# Autodesk Inventor assembly: Assembly
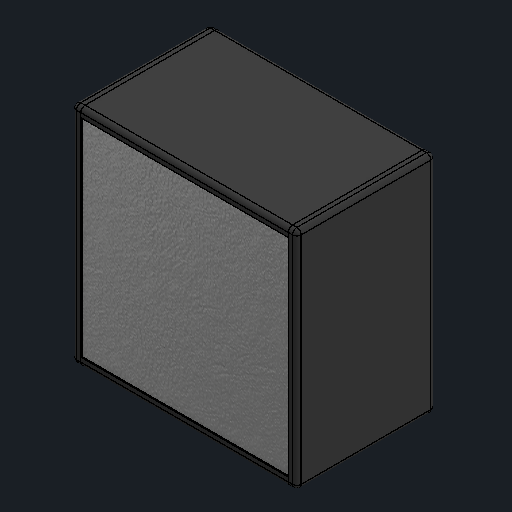
[picture p0: Inventor's stored thumbnail of the model, 512x512]
Saved by Autodesk Inventor 2026.2 (Build 302298000, 298)
## iProperties
Created: 2026-06-16
Part Number: Assembly
Document SubType Name: Assembly
Designer: JoshuaEah
Author: JoshuaEah
## Documents named in this file (18)
- C:\Users\JoshuaEah\Documents\GitHub\Designed-Trinkets\Guitar\110 Guitar Cab\Assembly.iam
- C:\Users\JoshuaEah\Documents\GitHub\Designed-Trinkets\Guitar\110 Guitar Cab\Wood Cuts\Bracing.iam
- C:\Users\JoshuaEah\Documents\GitHub\Designed-Trinkets\Guitar\110 Guitar Cab\Wood Cuts\Front Baffle.ipt
- C:\Users\JoshuaEah\Documents\GitHub\Designed-Trinkets\Guitar\110 Guitar Cab\Wood Cuts\Grille.ipt
- C:\Users\JoshuaEah\Documents\GitHub\Designed-Trinkets\Guitar\110 Guitar Cab\Sheet Metal\Jack Plate.ipt
- C:\Users\JoshuaEah\Documents\GitHub\Designed-Trinkets\Guitar\110 Guitar Cab\Hardware\Grill Cloth.ipt
- C:\Users\JoshuaEah\Documents\GitHub\Designed-Trinkets\Guitar\110 Guitar Cab\Wood Cuts\Top Panel.ipt
- C:\Users\JoshuaEah\Documents\GitHub\Designed-Trinkets\Guitar\110 Guitar Cab\Wood Cuts\Bottom Panel.ipt
- C:\Users\JoshuaEah\Documents\GitHub\Designed-Trinkets\Guitar\110 Guitar Cab\Wood Cuts\Side Panel (Right).ipt
- C:\Users\JoshuaEah\Documents\GitHub\Designed-Trinkets\Guitar\110 Guitar Cab\Wood Cuts\Side Panel (Left).ipt
- C:\Users\JoshuaEah\Documents\GitHub\Designed-Trinkets\Guitar\110 Guitar Cab\Hardware\Switchcraft C11X Jack.ipt
- C:\Users\JoshuaEah\Documents\GitHub\Designed-Trinkets\Guitar\110 Guitar Cab\Hardware\Switchcraft C11X Washer.ipt
- C:\Users\JoshuaEah\Documents\GitHub\Designed-Trinkets\Guitar\110 Guitar Cab\Hardware\Switchcraft C11X Nut.ipt
- C:\Users\JoshuaEah\Documents\GitHub\Designed-Trinkets\Guitar\110 Guitar Cab\Hardware\No. 4x1in PH1 Wood Screw.ipt
- C:\Users\JoshuaEah\Documents\GitHub\Designed-Trinkets\Guitar\110 Guitar Cab\Wood Cuts\Back Panel (Top).ipt
- C:\Users\JoshuaEah\Documents\GitHub\Designed-Trinkets\Guitar\110 Guitar Cab\Wood Cuts\Back Panel (Bottom).ipt
- C:\Users\JoshuaEah\Documents\GitHub\Designed-Trinkets\Guitar\110 Guitar Cab\Sheet Metal\Name Plate.ipt
- C:\Users\JoshuaEah\Documents\GitHub\Designed-Trinkets\Guitar\110 Guitar Cab\Hardware\No. 6-32x0.5in FHCS PH2.ipt
## Components (32 placed, 17 different names)
1. Top Panel:1 — Mate:1, Flush:1, Flush:2, Mate:2, Flush:3, Flush:4, Flush:10, Mate:16, Flush:15
2. Bottom Panel:1 — Flush:5, Flush:6, Mate:3
3. Side Panel (Right):1 — Mate:1, Flush:1, Flush:2, Flush:5, Flush:6, Mate:3, Mate:17
4. Side Panel (Left):1 — Mate:2, Flush:3, Flush:4
5. Front Baffle — Mate:20, Flush:16, Flush:17, Mate:21, Flush:18, Flush:19
6. Bracing:1 [sub-assembly] — Flush:15, Mate:20, Flush:16, Flush:17
7. Bracing:2 [sub-assembly] — Flush:10, Mate:16, Mate:17, Mate:18, Flush:11, Flush:12, Mate:19, Flush:13, Flush:14
8. Back Panel (Top):1 — Mate:18, Flush:11, Flush:12, Insert:8, Insert:12, Insert:13
9. Jack Plate:1 — Insert:3, Insert:4, Insert:14
10. Back Panel (Bottom):1 — Mate:19, Flush:13, Flush:14, Insert:9, Insert:18
11. Name Plate:1 — Insert:17, Insert:18
12. Grille:1 — Mate:21, Flush:18, Flush:19, Rigid:1
13. Grill Cloth:1 — Rigid:1
14. Switchcraft C11X Jack:1 — Insert:3
15. Switchcraft C11X Washer:1 — Insert:4, Insert:5
16. Switchcraft C11X Nut:1 — Insert:5
17. No. 4x1in PH1 Wood Screw:1 — Insert:8
18. No. 4x1in PH1 Wood Screw:2
19. No. 4x1in PH1 Wood Screw:3
20. No. 4x1in PH1 Wood Screw:4
21. No. 6-32x0.5in FHCS PH2:1 — Insert:14, Insert:13
22. No. 6-32x0.5in FHCS PH2:2
23. No. 6-32x0.5in FHCS PH2:3 — Insert:12
24. No. 6-32x0.5in FHCS PH2:4
25. No. 4x1in PH1 Wood Screw:5 — Insert:9
26. No. 4x1in PH1 Wood Screw:6
27. No. 4x1in PH1 Wood Screw:7
28. No. 4x1in PH1 Wood Screw:8
29. No. 6-32x0.5in FHCS PH2:5 — Insert:17
30. No. 6-32x0.5in FHCS PH2:6
31. No. 6-32x0.5in FHCS PH2:7
32. No. 6-32x0.5in FHCS PH2:8
## Component patterns: Back Plate (Top) Mounting Screws (4 elements), Jack Plate Mounting Screws (4 elements), Back Plate (Bottom) Mounting Screws (4 elements), Name Plate Mounting Screws (4 elements)
## Relationships (40: Flush 16, Mate 13, Insert 10, WeldJoint 1)
- Mate:1: Top Panel:1 ↔ Side Panel (Right):1
- Flush:1: Top Panel:1 ↔ Side Panel (Right):1
- Flush:2: Top Panel:1 ↔ Side Panel (Right):1
- Mate:2: Top Panel:1 ↔ Side Panel (Left):1
- Flush:3: Top Panel:1 ↔ Side Panel (Left):1
- Flush:4: Top Panel:1 ↔ Side Panel (Left):1
- Flush:5: Bottom Panel:1 ↔ Side Panel (Right):1
- Flush:6: Bottom Panel:1 ↔ Side Panel (Right):1
- Mate:3: Bottom Panel:1 ↔ Side Panel (Right):1
- [Mate]: Side Panel (Right):1 ↔ Bracing:1
- [Mate]: Top Panel:1 ↔ Bracing:1
- [Mate]: Top Panel:1 ↔ Bracing:1
- [Mate]: Side Panel (Left):1 ↔ Bracing:1
- Flush:10 (12.7 mm): Top Panel:1 ↔ Bracing:2
- Mate:16: Top Panel:1 ↔ Bracing:2
- Mate:17: Side Panel (Right):1 ↔ Bracing:2
- Mate:18: Bracing:2 ↔ Back Panel (Top):1
- Flush:11: Bracing:2 ↔ Back Panel (Top):1
- Flush:12: Bracing:2 ↔ Back Panel (Top):1
- Mate:19: Bracing:2 ↔ Back Panel (Bottom):1
- Flush:13: Bracing:2 ↔ Back Panel (Bottom):1
- Flush:14: Bracing:2 ↔ Back Panel (Bottom):1
- Flush:15 (19.05 mm): Top Panel:1 ↔ Bracing:1
- Mate:20: Front Baffle ↔ Bracing:1
- Flush:16: Front Baffle ↔ Bracing:1
- Flush:17: Front Baffle ↔ Bracing:1
- Mate:21: Front Baffle ↔ Grille:1
- Flush:18: Front Baffle ↔ Grille:1
- Flush:19: Front Baffle ↔ Grille:1
- Rigid:1 [WeldJoint]: Grille:1 ↔ Grill Cloth:1
- Insert:3: Jack Plate:1 ↔ Switchcraft C11X Jack:1
- Insert:4: Jack Plate:1 ↔ Switchcraft C11X Washer:1
- Insert:5: Switchcraft C11X Washer:1 ↔ Switchcraft C11X Nut:1
- Insert:8: Back Panel (Top):1 ↔ No. 4x1in PH1 Wood Screw:1
- Insert:9: Back Panel (Bottom):1 ↔ No. 4x1in PH1 Wood Screw:5
- Insert:12: Back Panel (Top):1 ↔ No. 6-32x0.5in FHCS PH2:3
- Insert:13: Back Panel (Top):1 ↔ No. 6-32x0.5in FHCS PH2:1
- Insert:14: Jack Plate:1 ↔ No. 6-32x0.5in FHCS PH2:1
- Insert:17: Name Plate:1 ↔ No. 6-32x0.5in FHCS PH2:5
- Insert:18: Back Panel (Bottom):1 ↔ Name Plate:1
## Named parameters: Finish1_Area = 4147.81, Finish1_Thickness = 0.05 mm
note: some values were not read from the file. Shown as the stored number, unit unknown: "Finish1_Area".
